# Autodesk Inventor assembly: Giant-Snes-Gamepad
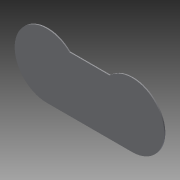
[picture p0: Inventor's stored thumbnail of the model, 180x180]
Saved by Autodesk Inventor 2014 SP1 (Build 180222100, 222)
## iProperties
Created: 2014-01-12
Part Number: Giant-Snes-Gamepad
Document SubType Name: Assembly
Designer: tuleu
Author: tuleu
## Documents named in this file (2)
- C:\Users\tuleu\Documents\giant-snes-gamepad\cad\Giant_Snes_Gamepad.iam
- C:\Users\tuleu\Documents\giant-snes-gamepad\cad\Base.ipt
## Components (2 placed, 1 different names)
1. Base:1 — Mate:1, Mate:2, Flush:1, Mate:3
2. Base:2 — Mate:1, Mate:2, Flush:1, Mate:3
## Relationships (4: Mate 3, Flush 1)
- Mate:1: Base:1 ↔ Base:2
- Mate:2: Base:1 ↔ Base:2
- Flush:1: Base:1 ↔ Base:2
- Mate:3: Base:1 ↔ Base:2
